# Autodesk Inventor assembly: Hoja Oculta 2
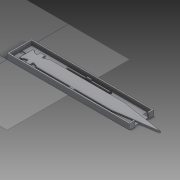
[picture p0: Inventor's stored thumbnail of the model, 180x180]
Saved by Autodesk Inventor 2011 (Build 150239000, 239)
## iProperties
Created: 2015-03-12
Part Number: Hoja Oculta 2
Document SubType Name: Assembly
Designer: amatiasq
Author: amatiasq
## Documents named in this file (3)
- C:\Users\amatiasq\Documents\GitHub\3D\Hoja Oculta Inventor\Piezas\Hoja Oculta 2.iam
- C:\Users\amatiasq\Documents\GitHub\3D\Hoja Oculta Inventor\Piezas\Base.ipt
- C:\Users\amatiasq\Documents\GitHub\3D\Hoja Oculta Inventor\Piezas\Hoja.ipt
## Components (2 placed, 2 different names)
1. Base:1 — Hoja-Base Inferior, Movimiento Hoja, Hoja-Base Lateral
2. Hoja:1 — Hoja-Base Inferior, Movimiento Hoja, Hoja-Base Lateral
## Relationships (3: Mate 3)
- Hoja-Base Inferior [Mate] (0.3 mm): Base:1 ↔ Hoja:1
- Movimiento Hoja [Mate]: Base:1 ↔ Hoja:1
- Hoja-Base Lateral [Mate] (0.3 mm): Base:1 ↔ Hoja:1
